# Autodesk Inventor assembly: ASY ДМФ 0100 Барабан v2.1
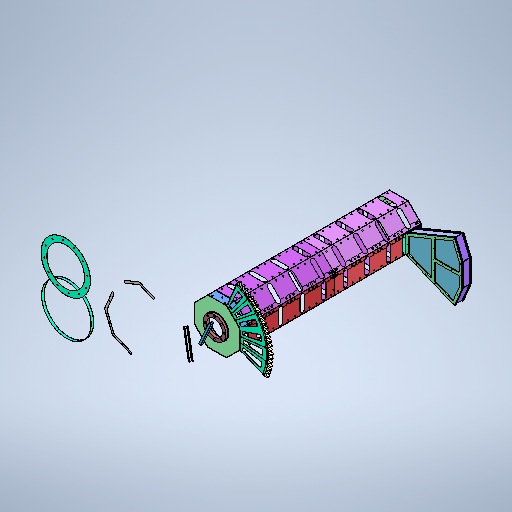
[picture p0: Inventor's stored thumbnail of the model, 512x512]
Saved by Autodesk Inventor 2026.2 (Build 302298010, 298A)
## iProperties
Created: 2024-04-28
Part Number: ASY ДМФ 0100 Барабан v2.1
Document SubType Name: Assembly
Designer: pokla
Author: pokla
## Documents named in this file (22)
- C:\Users\admin\Documents\Inventor\DMF-Disk-Micro-Filter\Барабан v2.1\ASY ДМФ 0100 Барабан v2.1.iam
- C:\Users\admin\Documents\Inventor\DMF-Disk-Micro-Filter\Барабан v2.1\DMF 01 21 Барабан торец НОС v2.1.ipt
- C:\Users\admin\Documents\Inventor\DMF-Disk-Micro-Filter\Барабан v2.1\DMF 01 13 Барабан Лист лев брт v2.1.ipt
- C:\Users\admin\Documents\Inventor\DMF-Disk-Micro-Filter\Барабан v2.1\DMF 01 14 Барабан Лист прав брт v2.1.ipt
- C:\Users\admin\Documents\Inventor\DMF-Disk-Micro-Filter\Барабан v2.1\DMF 01 31 Барабан Опорное кольцо НОС v2.1.ipt
- C:\Users\admin\Documents\Inventor\DMF-Disk-Micro-Filter\Барабан v2.1\DMF 01 17 опора крышки v2.1.ipt
- C:\Users\admin\Documents\Inventor\DMF-Disk-Micro-Filter\Барабан v2.1\DMF 000 размеры v2.1.ipt
- C:\Users\admin\Documents\Inventor\DMF-Disk-Micro-Filter\Барабан v2.1\DMF 01 12 Барабан усилитель v2.1.ipt
- C:\Users\admin\Documents\Inventor\DMF-Disk-Micro-Filter\Барабан v2.1\ASY DMF 010 cap v2.1.iam
- C:\Users\admin\Documents\Inventor\DMF-Disk-Micro-Filter\Барабан v2.1\DMF 01 32 Барабан Опорное кольцо КОРМА v2.1.ipt
- C:\Users\admin\Documents\Inventor\DMF-Disk-Micro-Filter\Барабан v2.1\DMF 01 22 Барабан торец КОРМА v2.1.ipt
- C:\Users\admin\Documents\Inventor\DMF-Disk-Micro-Filter\Барабан v2.1\ASY DMF filter package v2.1.iam
- C:\Users\admin\Documents\Inventor\DMF-Disk-Micro-Filter\Барабан v2.1\DMF 2.1 01 45 Gear ring 5.ipt
- C:\Users\admin\Documents\Inventor\DMF-Disk-Micro-Filter\Барабан v2.1\DMF 2.1 01 46 Gear axis wheel 6.ipt
- C:\Users\admin\Documents\Inventor\DMF-Disk-Micro-Filter\Барабан v2.1\DMF 01 13 Барабан усилитель v2.1.ipt
- C:\Users\admin\Documents\Inventor\DMF-Disk-Micro-Filter\Барабан v2.1\DMF 01 15 drum sheet 1.ipt
- C:\Users\admin\Documents\Inventor\DMF-Disk-Micro-Filter\ДМФ 01 12 Барабан усилитель.ipt
- C:\Users\admin\Documents\Inventor\DMF-Disk-Micro-Filter\ДМФ 01 15 Барабан усилитель борта.ipt
- C:\Users\admin\Documents\Inventor\DMF-Disk-Micro-Filter\Барабан v2.1\DMF 01 11 cylinder sheet cap v2.1.ipt
- C:\Users\admin\Documents\Inventor\DMF-Disk-Micro-Filter\ContentCenter\en-US\DIN 913\DIN 913 - M12 x 20.ipt
- C:\Users\admin\Documents\Inventor\DMF-Disk-Micro-Filter\Барабан v2.1\DMF 01 11 cylinder sheet cap v2.1_CPY.ipt
- C:\Users\admin\Documents\Inventor\DMF-Disk-Micro-Filter\Барабан v2.1\DMF 01 21 Барабан торец НОС v2.1_наруж.ipt
## Components (34 placed, 26 different names)
1. DMF 000 размеры v2.1.ipt:1
2. DMF 01 21 Барабан торец НОС v2.1.ipt:1 — Rigid:115, Rigid:120
3. DMF 01 31 Барабан Опорное кольцо НОС v2.1.ipt:1 — Rigid:125
4. DMF 01 32 Барабан Опорное кольцо КОРМА v2.1.ipt:1 — Rigid:126
5. DMF 01 22 Барабан торец КОРМА v2.1.ipt:1 — Rigid:51, Mate:37, Rigid:97, Mate:46, Mate:50, Flush:36, Mate:51, Rigid:126, Mate:54
6. DMF 01 13 Барабан Лист лев брт v2.1.ipt:1 — Rigid:51, Rigid:98
7. DMF 01 14 Барабан Лист прав брт v2.1.ipt:1 — Mate:54, Mate:55, Mate:56
8. DMF 01 17 опора крышки v2.1.ipt:1 — Mate:37, Mate:46, Mate:47, Mate:48, Rigid:112
9. DMF 01 11 cylinder sheet cap v2.1.ipt:1 — Mate:47, Rotational:1, Rigid:122, Mate:55, Mate:56
10. ASY DMF 010 cap v2.1.iam:1 [sub-assembly] — Mate:57, Mate:58, Flush:37
11. DMF 2.1 01 45 Gear ring 5.ipt:1
12. DMF 2.1 01 46 Gear axis wheel 6.ipt:1
13. ДМФ 01 12 Барабан усилитель.ipt:2
14. ДМФ 01 15 Барабан усилитель борта.ipt:4
15. DMF 01 12 Барабан усилитель v2.1.ipt:2
16. DMF 01 13 Барабан усилитель v2.1.ipt:2
17. DMF 01 13 Барабан Лист лев брт v2.1:2 — Rigid:97, Rigid:99, Mate:48
18. DMF 01 13 Барабан Лист лев брт v2.1:3 — Rigid:98
19. DMF 01 13 Барабан Лист лев брт v2.1:4 — Rigid:99, Rigid:115
20. DMF 01 17 опора крышки v2.1:4 — Rigid:112
21. DMF 01 21 Барабан торец НОС v2.1:3 — Rigid:120, Rigid:127, Rigid:128, Rigid:130, Rigid:131, Rigid:132, Rigid:133, Rigid:134, Rigid:135
22. DIN 913 M12 x 20:1 — Rotational:1
23. DMF 01 11 cylinder sheet cap v2.1:2 — Rigid:122, Rigid:123
24. ASY DMF filter package v2.1.iam:1 [sub-assembly]
25. DMF 01 11 cylinder sheet cap v2.1_CPY:1 — Rigid:123
26. DMF 01 21 Барабан торец НОС v2.1_наруж:1 — Rigid:125, Rigid:129, Flush:37
27. DMF 01 15 drum sheet 1:8 — Rigid:135
28. DMF 01 15 drum sheet 1:7 — Rigid:133
29. DMF 01 15 drum sheet 1:6 — Rigid:134
30. DMF 01 15 drum sheet 1:5 — Rigid:132
31. DMF 01 15 drum sheet 1:4 — Rigid:131, Mate:58
32. DMF 01 15 drum sheet 1:3 — Rigid:130, Mate:57
33. DMF 01 15 drum sheet 1:2 — Rigid:128
34. DMF 01 15 drum sheet 1.ipt:1 — Rigid:127, Rigid:129
## Relationships (38: WeldJoint 21, Mate 12, Flush 4, RevoluteJoint 1)
- Rigid:51 [WeldJoint]: DMF 01 22 Барабан торец КОРМА v2.1.ipt:1 ↔ DMF 01 13 Барабан Лист лев брт v2.1.ipt:1
- Mate:37: DMF 01 22 Барабан торец КОРМА v2.1.ipt:1 ↔ DMF 01 17 опора крышки v2.1.ipt:1
- [Mate]: DMF 01 22 Барабан торец КОРМА v2.1.ipt:1 ↔ DMF 01 11 cylinder sheet cap v2.1.ipt:1
- [Flush]: DMF 01 22 Барабан торец КОРМА v2.1.ipt:1 ↔ DMF 01 11 cylinder sheet cap v2.1.ipt:1
- [Flush]: DMF 01 22 Барабан торец КОРМА v2.1.ipt:1 ↔ DMF 01 11 cylinder sheet cap v2.1.ipt:1
- [WeldJoint]: DMF 01 11 cylinder sheet cap v2.1.ipt:1 ↔ ASY DMF filter package v2.1.iam:1
- Rigid:97 [WeldJoint]: DMF 01 22 Барабан торец КОРМА v2.1.ipt:1 ↔ DMF 01 13 Барабан Лист лев брт v2.1:2
- Rigid:98 [WeldJoint]: DMF 01 13 Барабан Лист лев брт v2.1.ipt:1 ↔ DMF 01 13 Барабан Лист лев брт v2.1:3
- Rigid:99 [WeldJoint]: DMF 01 13 Барабан Лист лев брт v2.1:2 ↔ DMF 01 13 Барабан Лист лев брт v2.1:4
- Mate:46: DMF 01 22 Барабан торец КОРМА v2.1.ipt:1 ↔ DMF 01 17 опора крышки v2.1.ipt:1
- Mate:47: DMF 01 17 опора крышки v2.1.ipt:1 ↔ DMF 01 11 cylinder sheet cap v2.1.ipt:1
- Mate:48: DMF 01 17 опора крышки v2.1.ipt:1 ↔ DMF 01 13 Барабан Лист лев брт v2.1:2
- Rigid:112 [WeldJoint]: DMF 01 17 опора крышки v2.1.ipt:1 ↔ DMF 01 17 опора крышки v2.1:4
- Mate:50: DMF 01 22 Барабан торец КОРМА v2.1.ipt:1
- Flush:36: DMF 01 22 Барабан торец КОРМА v2.1.ipt:1
- Mate:51: DMF 01 22 Барабан торец КОРМА v2.1.ipt:1
- Rigid:115 [WeldJoint]: DMF 01 21 Барабан торец НОС v2.1.ipt:1 ↔ DMF 01 13 Барабан Лист лев брт v2.1:4
- Rigid:120 [WeldJoint]: DMF 01 21 Барабан торец НОС v2.1.ipt:1 ↔ DMF 01 21 Барабан торец НОС v2.1:3
- Rotational:1 [RevoluteJoint]: DMF 01 11 cylinder sheet cap v2.1.ipt:1 ↔ DIN 913 M12 x 20:1
- Rigid:122 [WeldJoint]: DMF 01 11 cylinder sheet cap v2.1.ipt:1 ↔ DMF 01 11 cylinder sheet cap v2.1:2
- Rigid:123 [WeldJoint]: DMF 01 11 cylinder sheet cap v2.1:2 ↔ DMF 01 11 cylinder sheet cap v2.1_CPY:1
- Rigid:125 [WeldJoint]: DMF 01 31 Барабан Опорное кольцо НОС v2.1.ipt:1 ↔ DMF 01 21 Барабан торец НОС v2.1_наруж:1
- Rigid:126 [WeldJoint]: DMF 01 32 Барабан Опорное кольцо КОРМА v2.1.ipt:1 ↔ DMF 01 22 Барабан торец КОРМА v2.1.ipt:1
- Mate:54: DMF 01 22 Барабан торец КОРМА v2.1.ipt:1 ↔ DMF 01 14 Барабан Лист прав брт v2.1.ipt:1
- Mate:55: DMF 01 14 Барабан Лист прав брт v2.1.ipt:1 ↔ DMF 01 11 cylinder sheet cap v2.1.ipt:1
- Mate:56: DMF 01 14 Барабан Лист прав брт v2.1.ipt:1 ↔ DMF 01 11 cylinder sheet cap v2.1.ipt:1
- Rigid:127 [WeldJoint]: DMF 01 21 Барабан торец НОС v2.1:3 ↔ DMF 01 15 drum sheet 1.ipt:1
- Rigid:128 [WeldJoint]: DMF 01 21 Барабан торец НОС v2.1:3 ↔ DMF 01 15 drum sheet 1:2
- Rigid:129 [WeldJoint]: DMF 01 21 Барабан торец НОС v2.1_наруж:1 ↔ DMF 01 15 drum sheet 1.ipt:1
- Rigid:130 [WeldJoint]: DMF 01 21 Барабан торец НОС v2.1:3 ↔ DMF 01 15 drum sheet 1:3
- Rigid:131 [WeldJoint]: DMF 01 21 Барабан торец НОС v2.1:3 ↔ DMF 01 15 drum sheet 1:4
- Rigid:132 [WeldJoint]: DMF 01 21 Барабан торец НОС v2.1:3 ↔ DMF 01 15 drum sheet 1:5
- Rigid:133 [WeldJoint]: DMF 01 21 Барабан торец НОС v2.1:3 ↔ DMF 01 15 drum sheet 1:7
- Rigid:134 [WeldJoint]: DMF 01 21 Барабан торец НОС v2.1:3 ↔ DMF 01 15 drum sheet 1:6
- Rigid:135 [WeldJoint]: DMF 01 21 Барабан торец НОС v2.1:3 ↔ DMF 01 15 drum sheet 1:8
- Mate:57: ASY DMF 010 cap v2.1.iam:1 ↔ DMF 01 15 drum sheet 1:3
- Mate:58: ASY DMF 010 cap v2.1.iam:1 ↔ DMF 01 15 drum sheet 1:4
- Flush:37: ASY DMF 010 cap v2.1.iam:1 ↔ DMF 01 21 Барабан торец НОС v2.1_наруж:1
